# Autodesk Inventor assembly: фуллл
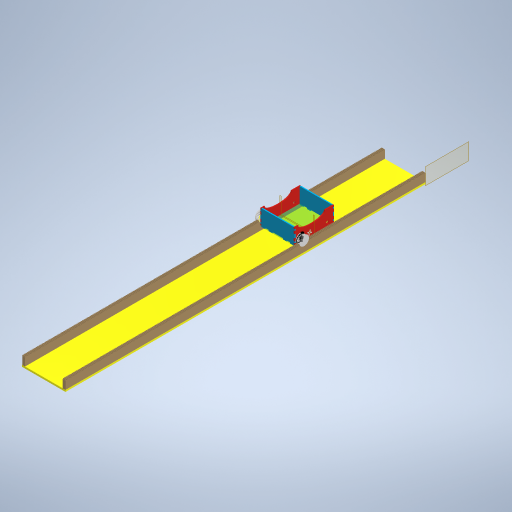
[picture p0: Inventor's stored thumbnail of the model, 512x512]
Saved by Autodesk Inventor 2024.2 (Build 282272000, 272)
## iProperties
Created: 2025-11-20
Part Number: фуллл
Document SubType Name: Assembly
Designer: Zakhar
Mass: 774.945 g
Surface Area: 2621.06 cm^2
Volume: 774.945 cm^3
Density: 1 g/cm^3
Author: Zakhar
## Documents named in this file (11)
- C:\Users\Zakhar\Documents\Artist\3D\Робот.iam
- C:\Users\Zakhar\Documents\Artist\3D\NEMA17 42-40.ipt
- C:\Users\Zakhar\Documents\Artist\3D\боковая стенка.ipt
- C:\Users\Zakhar\Documents\Artist\3D\Муфта.ipt
- C:\Users\Zakhar\Documents\Artist\3D\передняя стенка.ipt
- C:\Users\Zakhar\Documents\Artist\3D\Шест.ipt
- C:\Users\Zakhar\Documents\Artist\3D\Нижняя крышка.ipt
- C:\Users\Zakhar\Documents\Artist\3D\крепление подшипника_1.ipt
- C:\Users\Zakhar\Documents\Artist\3D\Муфта_MIR.ipt
- C:\Users\Zakhar\Documents\Artist\3D\Шест_MIR.ipt
- C:\Users\Zakhar\Documents\Artist\3D\полигон етз\полигон етз.ipt
## Components (13 placed, 10 different names)
1. NEMA17 42-40:1 — Жесткий:5, С поворотом:2
2. боковая стенка:1 — Жесткий:2, Жесткий:7, Симметрия:1
3. Муфта:1 — С поворотом:1, Жесткий:8
4. передняя стенка:1 — Жесткий:3
5. Шест:1 — Жесткий:8, Заподлицо:1
6. боковая стенка:2 — Жесткий:1, Жесткий:3, Жесткий:5, Совмещение:2, Симметрия:1
7. передняя стенка:2 — Жесткий:1, Жесткий:2, Жесткий:6
8. Нижняя крышка:1 — Жесткий:6, Совмещение:1
9. NEMA17 42-40:2 — Жесткий:7, С поворотом:1
10. крепление подшипника_1:1
11. Муфта_MIR:1 — Жесткий:9, С поворотом:2
12. Шест_MIR:1 — Жесткий:9
13. полигон етз:1 — Совмещение:3, Заподлицо:1
## Relationships (15: WeldJoint 8, Mate 3, RevoluteJoint 2, Symmetry 1, Flush 1)
- Жесткий:1 [WeldJoint]: боковая стенка:2 ↔ передняя стенка:2
- Жесткий:2 [WeldJoint]: боковая стенка:1 ↔ передняя стенка:2
- Жесткий:3 [WeldJoint]: передняя стенка:1 ↔ боковая стенка:2
- Жесткий:5 [WeldJoint]: NEMA17 42-40:1 ↔ боковая стенка:2
- Жесткий:6 [WeldJoint]: передняя стенка:2 ↔ Нижняя крышка:1
- Совмещение:1 [Mate]: Нижняя крышка:1
- Совмещение:2 [Mate]: боковая стенка:2
- Жесткий:7 [WeldJoint]: боковая стенка:1 ↔ NEMA17 42-40:2
- С поворотом:1 [RevoluteJoint]: Муфта:1 ↔ NEMA17 42-40:2
- Жесткий:8 [WeldJoint]: Муфта:1 ↔ Шест:1
- Симметрия:1 [Symmetry]: боковая стенка:1 ↔ боковая стенка:2
- Жесткий:9 [WeldJoint] (-4 mm): Муфта_MIR:1 ↔ Шест_MIR:1
- С поворотом:2 [RevoluteJoint]: NEMA17 42-40:1 ↔ Муфта_MIR:1
- Совмещение:3 [Mate] (-40.826 mm): полигон етз:1
- Заподлицо:1 [Flush] (4 mm): Шест:1 ↔ полигон етз:1
